# Autodesk Inventor assembly: winch assembly
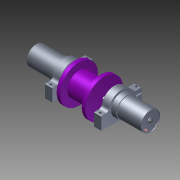
[picture p0: Inventor's stored thumbnail of the model, 180x180]
Saved by Autodesk Inventor 2015 SP1 (Build 190203100, 203)
## iProperties
Created: 2014-10-15
Part Number: winch assembly
Document SubType Name: Assembly
Designer: aumccarville
Author: aumccarville
## Documents named in this file (4)
- C:\Users\datenney\Documents\GitHub\CAD\winch assembly.iam
- C:\Users\datenney\Documents\GitHub\CAD\2014_robotComplete\Imported Components\motor mount\motor mount.ipt
- C:\Users\datenney\Documents\GitHub\CAD\2014_robotComplete\Imported Components\motor\motor.iam
- C:\Users\datenney\Documents\GitHub\CAD\2014_robotComplete\Spool.ipt
## Components (5 placed, 3 different names)
1. motor mount:1 — Mate:1, Flush:2, Flush:3, Flush:4
2. motor mount:2 — Flush:1, Mate:2, Flush:3, Flush:4
3. Spool:1 — Mate:3, Mate:4, Mate:5, Mate:6
4. motor:1 [sub-assembly] — Mate:1, Flush:2, Mate:4, Mate:5
5. motor:2 [sub-assembly] — Flush:1, Mate:2, Mate:3, Mate:6
## Relationships (10: Mate 6, Flush 4)
- Mate:1: motor mount:1 ↔ motor:1
- Flush:1: motor mount:2 ↔ motor:2
- Mate:2: motor mount:2 ↔ motor:2
- Flush:2: motor mount:1 ↔ motor:1
- Mate:3: Spool:1 ↔ motor:2
- Mate:4: Spool:1 ↔ motor:1
- Mate:5 (-19.05 mm): Spool:1 ↔ motor:1
- Mate:6 (-19.05 mm): Spool:1 ↔ motor:2
- Flush:3: motor mount:1 ↔ motor mount:2
- Flush:4: motor mount:1 ↔ motor mount:2
